# Autodesk Inventor assembly: body_new
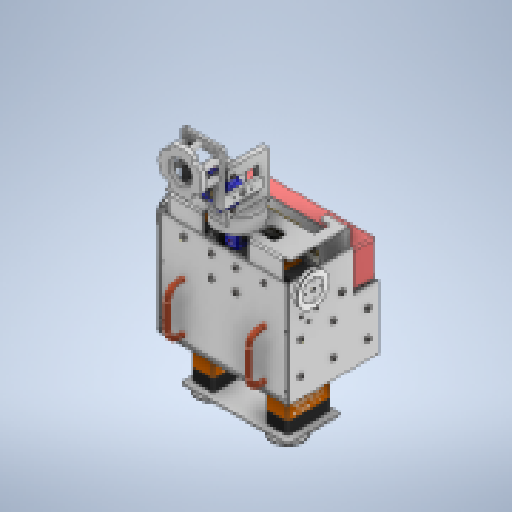
[picture p0: Inventor's stored thumbnail of the model, 512x512]
Saved by Autodesk Inventor 2027.1 (Build 311270010, 270A)
## iProperties
Created: 2025-05-30
Part Number: body_new
Document SubType Name: Assembly
Designer: chris
Author: chris
## Documents named in this file (30)
- C:\Users\chanh\Documents\RHp_Humanoid_ver1\Total\body_new.iam
- C:\Users\chanh\Documents\RHp_Humanoid_ver1\Part_Body\Frame\Body\body_main_frame.ipt
- C:\Users\chanh\Documents\RHp_Humanoid_ver1\Part_Body\Frame\Body\body_back_frame.ipt
- C:\Users\chanh\Documents\RHp_Humanoid_ver1\Part_Body\Frame\Body\body_front_frame.ipt
- C:\Users\chanh\Documents\RHp_Humanoid_ver1\Part_Body\Frame\Body\body_middle_frame.ipt
- C:\Users\chanh\Documents\RHp_Humanoid_ver1\Part_Body\Frame\Body\body_motor_L_frame.ipt
- C:\Users\chanh\Documents\RHp_Humanoid_ver1\Part_Body\Frame\Body\body_motor_R_frame.ipt
- C:\Users\chanh\Documents\RHp_Humanoid_ver1\Part_Body\Other Parts\Servo_Driver.ipt
- C:\Users\chanh\Documents\RHp_Humanoid_ver1\Part_Body\Other Parts\Battery_Pack.ipt
- C:\Users\chanh\Documents\RHp_Humanoid_ver1\Part_Body\Other Parts\jetson_orin_super.ipt
- C:\Users\chanh\Documents\RHp_Humanoid_ver1\Part_Body\Frame\Body\body_bottom_frame.ipt
- C:\Users\chanh\Documents\RHp_Humanoid_ver1\Part_Body\Other Parts\frame_motor_support_top_R.ipt
- C:\Users\chanh\Documents\RHp_Humanoid_ver1\Part_Body\Other Parts\frame_motor_support_top_L.ipt
- C:\Users\chanh\Documents\RHp_Humanoid_ver1\Part_Body\Bolt, Bearing, Nut, Washer\2030 Teflon Sheet.ipt
- C:\Users\chanh\Documents\RHp_Humanoid_ver1\Part_Body\Other Parts\frame_support.ipt
- C:\Users\chanh\Documents\RHp_Humanoid_ver1\Part_Body\HTD-45H, Horn (Silver)\HTD-45H\HTD-45H.ipt
- C:\Users\chanh\Documents\RHp_Humanoid_ver1\Part_Body\Other Parts\frame_motor_support_bottom_L.ipt
- C:\Users\chanh\Documents\RHp_Humanoid_ver1\Part_Body\Other Parts\frame_motor_support_bottom_R.ipt
- C:\Users\chanh\Documents\RHp_Humanoid_ver1\Part_Body\Bolt, Bearing, Nut, Washer\M3x6 Bolt.ipt
- C:\Users\chanh\Documents\RHp_Humanoid_ver1\Part_Body\Bolt, Bearing, Nut, Washer\M3 Nut.ipt
- C:\Users\chanh\Documents\RHp_Humanoid_ver1\Part_Body\Bolt, Bearing, Nut, Washer\M2x4 Bolt.ipt
- C:\Users\chanh\Documents\RHp_Humanoid_ver1\Part_Body\Bolt, Bearing, Nut, Washer\M2x6 Bolt.ipt
- C:\Users\chanh\Documents\RHp_Humanoid_ver1\Part_Body\Bolt, Bearing, Nut, Washer\M2x35 Bolt.ipt
- C:\Users\chanh\Documents\RHp_Humanoid_ver1\Part_Body\HTD-45H, Horn (Silver)\HTD-45H\M2x32.ipt
- C:\Users\chanh\Documents\RHp_Humanoid_ver1\Part_Body\HTD-45H, Horn (Silver)\Horn\Top Horn.ipt
- C:\Users\chanh\Documents\RHp_Humanoid_ver1\Part_Body\Frame\Body\body_top_frame2.ipt
- C:\Users\chanh\Documents\RHp_Humanoid_ver1\Part_Body\Other Parts\head\SG90 - Micro Servo 9g - Tower Pro\SG90 - Micro Servo 9g - Tower Pro\SG90 - Micro Servo 9g - Tower Pro - bottom.iam
- C:\Users\chanh\Documents\RHp_Humanoid_ver1\Part_Body\Other Parts\head\head_bottom.ipt
- C:\Users\chanh\Documents\RHp_Humanoid_ver1\Part_Body\Other Parts\head\head_top.ipt
- C:\Users\chanh\Documents\RHp_Humanoid_ver1\Part_Body\Other Parts\head\SG90 - Micro Servo 9g - Tower Pro\SG90 - Micro Servo 9g - Tower Pro\SG90 - Micro Servo 9g - Tower Pro - top.iam
## Components (171 placed, 29 different names)
1. head_bottom:1 — Rigid:157, Mate:93, Mate:94, Flush:38
2. head_top:1 — Rigid:158
3. SG90 - Micro Servo 9g - Tower Pro - top:1 [sub-assembly] — Mate:93, Mate:94, Flush:38, Rigid:158
4. body_main_frame:1 — Mate:3, Flush:2, Mate:4, Mate:5, Flush:3, Flush:4, Mate:6, Flush:5, Mate:8, Mate:10, Mate:16, Mate:18, Flush:13, Mate:30, Flush:30, Flush:31, Mate:46, Mate:47, Mate:48, Mate:49, Mate:50, Mate:51, Mate:64, Mate:66, Mate:68, Flush:34, Flush:35, Mate:69, Flush:36, Flush:37, Rigid:25, Rigid:26, Rigid:29, Rigid:30, Rigid:33, Rigid:34, Rigid:35, Rigid:36, Rigid:65, Rigid:66, Rigid:67, Rigid:68, Rigid:73, Rigid:74, Rigid:75, Rigid:76, Rigid:77, Rigid:78, Rigid:99, Rigid:100, Rigid:101, Rigid:102, Rigid:103, Rigid:104, Rigid:105, Rigid:106, Rigid:107, Rigid:108, Rigid:109, Rigid:110, Rigid:145, Rigid:147
5. body_middle_frame:1 — Mate:6, Flush:5, Flush:6, Mate:17, Mate:28, Flush:29, Mate:29, Mate:65, Flush:32, Flush:33, Mate:67, Rigid:9, Rigid:10, Rigid:11, Rigid:12, Rigid:13, Rigid:14, Rigid:15, Rigid:16, Rigid:27, Rigid:28, Rigid:31, Rigid:32
6. body_front_frame:1 — Mate:5, Flush:3, Flush:4, Flush:6, Mate:7, Flush:7, Mate:9, Flush:8, Mate:58, Mate:59, Mate:60, Mate:61, Mate:62, Mate:63, Rigid:17, Rigid:18, Rigid:19, Rigid:20, Rigid:49, Rigid:50, Rigid:51, Rigid:52, Rigid:57, Rigid:58, Rigid:59, Rigid:60, Rigid:69, Rigid:70, Rigid:71, Rigid:72, Rigid:149, Rigid:151, Rigid:152
7. body_back_frame:1 — Mate:3, Flush:2, Mate:4, Mate:19, Mate:52, Mate:53, Mate:54, Mate:55, Mate:56, Mate:57, Rigid:37, Rigid:38, Rigid:39, Rigid:40, Rigid:61, Rigid:62, Rigid:63, Rigid:64
8. body_top_frame2:1 — Rigid:152, Rigid:153, Rigid:154, Rigid:155, Rigid:156, Mate:89, Mate:91, Mate:95, Mate:96
9. body_bottom_frame:1 — Mate:80, Mate:81, Mate:82, Mate:83, Mate:84, Mate:85, Mate:86, Mate:87, Mate:88, Rigid:111, Rigid:112, Rigid:113, Rigid:114, Rigid:115, Rigid:116
10. Servo_Driver:1 — Mate:16, Mate:17, Mate:18, Rigid:1, Rigid:2, Rigid:3, Rigid:4
11. Battery_Pack:1 — Mate:19, Flush:13, Mate:89
12. jetson_orin_super:1 — Mate:28, Flush:29, Mate:29
13. SG90 - Micro Servo 9g - Tower Pro - bottom:1 [sub-assembly] — Mate:91, Rigid:157, Mate:95, Mate:96
14. HTD-45H:1 — Mate:69, Flush:36, Flush:37, Mate:81, Rigid:127, Rigid:128, Rotational:8
15. HTD-45H:2 — Mate:68, Flush:34, Flush:35, Mate:80, Mate:82, Rigid:125, Rigid:126, Rotational:7
16. HTD-45H:3 — Mate:66, Flush:33, Mate:67, Rigid:129, Rigid:130, Rotational:5
17. HTD-45H:4 — Mate:64, Mate:65, Flush:32, Rigid:131, Rigid:132, Rotational:6
18. Top Horn:5 — Rotational:5
19. Top Horn:7 — Rotational:6
20. 2030 Teflon Sheet:1 — Insert:2, Insert:9
21. 2030 Teflon Sheet:2 — Insert:2
22. 2030 Teflon Sheet:3 — Insert:4, Insert:10
23. 2030 Teflon Sheet:4 — Insert:4
24. frame_motor_support_top_R:1 — Mate:46, Mate:47, Mate:48, Rigid:81, Rigid:84, Rigid:85, Rigid:86, Insert:10
25. frame_motor_support_top_L:1 — Mate:49, Mate:50, Mate:51, Rigid:79, Rigid:80, Rigid:82, Rigid:83, Insert:9
26. body_motor_R_frame:1 — Mate:9, Mate:10, Flush:8, Rigid:5, Rigid:7, Rigid:22, Rigid:24, Rigid:53, Rigid:54, Rigid:87, Rigid:88, Rigid:89, Rigid:90, Rigid:91, Rigid:92
27. body_motor_L_frame:1 — Mate:7, Flush:7, Mate:8, Rigid:6, Rigid:8, Rigid:21, Rigid:23, Rigid:55, Rigid:56, Rigid:93, Rigid:94, Rigid:95, Rigid:96, Rigid:97, Rigid:98
28. M3x6 Bolt:9 — Rigid:17
29. M3x6 Bolt:10 — Rigid:20
30. M3x6 Bolt:11 — Rigid:18
31. M3x6 Bolt:12 — Rigid:19
32. M3x6 Bolt:13 — Rigid:29
33. M3x6 Bolt:14 — Rigid:30
34. M3x6 Bolt:15 — Rigid:26
35. M3x6 Bolt:16 — Rigid:25
36. M3 Nut:9 — Rigid:24
37. M3 Nut:10 — Rigid:23
38. M3 Nut:11 — Rigid:22
39. M3 Nut:12 — Rigid:21
40. M3 Nut:13 — Rigid:31
41. M3 Nut:14 — Rigid:32
42. M3 Nut:15 — Rigid:27
43. M3 Nut:16 — Rigid:28
44. M3x6 Bolt:1 — Rigid:4
45. M3x6 Bolt:2 — Rigid:3
46. M3x6 Bolt:3 — Rigid:2
47. M3x6 Bolt:4 — Rigid:1
48. M3x6 Bolt:5 — Rigid:5
49. M3x6 Bolt:6 — Rigid:6
50. M3x6 Bolt:7 — Rigid:7
51. M3x6 Bolt:8 — Rigid:8
52. M3 Nut:1 — Rigid:9
53. M3 Nut:2 — Rigid:10
54. M3 Nut:3 — Rigid:11
55. M3 Nut:4 — Rigid:12
56. M3 Nut:5 — Rigid:13
57. M3 Nut:6 — Rigid:14
58. M3 Nut:7 — Rigid:15
59. M3 Nut:8 — Rigid:16
60. frame_support:3 — Mate:59, Mate:61, Mate:63
61. frame_support:4 — Mate:58, Mate:60, Mate:62
62. M3x6 Bolt:37 — Rigid:66
63. M3x6 Bolt:38 — Rigid:65
64. M3x6 Bolt:39 — Rigid:68
65. M3x6 Bolt:40 — Rigid:67
66. M3 Nut:29 — Rigid:69
67. M3 Nut:30 — Rigid:70
68. M3 Nut:31 — Rigid:71
69. M3 Nut:32 — Rigid:72
70. M3x6 Bolt:29 — Rigid:57
71. M3x6 Bolt:30 — Rigid:58
72. M3x6 Bolt:31 — Rigid:60
73. M3x6 Bolt:32 — Rigid:59
74. M3x6 Bolt:25 — Rigid:49
75. M3x6 Bolt:26 — Rigid:51
76. M3x6 Bolt:27 — Rigid:50
77. M3x6 Bolt:28 — Rigid:52
78. M3 Nut:25 — Rigid:53
79. M3 Nut:26 — Rigid:55
80. M3 Nut:27 — Rigid:54
81. M3 Nut:28 — Rigid:56
82. frame_support:1 — Mate:52, Mate:53, Mate:54
83. frame_support:2 — Mate:55, Mate:56, Mate:57
84. M3x6 Bolt:33 — Rigid:61
85. M3x6 Bolt:34 — Rigid:62
86. M3x6 Bolt:35 — Rigid:64
87. M3x6 Bolt:36 — Rigid:63
88. M3x6 Bolt:17 — Rigid:33
89. M3x6 Bolt:18 — Rigid:35
90. M3x6 Bolt:19 — Rigid:34
91. M3x6 Bolt:20 — Rigid:36
92. M3 Nut:17 — Rigid:37
93. M3 Nut:18 — Rigid:38
94. M3 Nut:19 — Rigid:39
95. M3 Nut:20 — Rigid:40
96. M3x6 Bolt:45 — Rigid:147
97. M3x6 Bolt:46 — Rigid:151
98. M3x6 Bolt:47 — Rigid:145
99. M3x6 Bolt:48 — Rigid:149
100. M3 Nut:41 — Rigid:156
101. M3 Nut:42 — Rigid:153
102. M3 Nut:43 — Rigid:155
103. M3 Nut:44 — Rigid:154
104. frame_motor_support_bottom_R:1 — Mate:83, Mate:84, Mate:85, Rigid:119, Rigid:120, Rigid:121, Rigid:122, Insert:12
105. frame_motor_support_bottom_L:1 — Mate:86, Mate:87, Mate:88, Rigid:117, Rigid:118, Rigid:123, Rigid:124, Insert:11
106. 2030 Teflon Sheet:5 — Insert:8
107. 2030 Teflon Sheet:6 — Insert:8, Insert:11
108. 2030 Teflon Sheet:7 — Insert:6
109. 2030 Teflon Sheet:8 — Insert:6, Insert:12
110. Top Horn:6 — Rotational:7
111. Top Horn:8 — Rotational:8
112. M2x32:7 — Rigid:132
113. M2x32:8 — Rigid:131
114. M2x4 Bolt:7 — Rigid:87
115. M2x4 Bolt:8 — Rigid:89
116. M2x4 Bolt:9 — Rigid:91
117. M2x4 Bolt:10 — Rigid:88
118. M2x4 Bolt:11 — Rigid:90
119. M2x4 Bolt:12 — Rigid:92
120. M2x4 Bolt:4 — Rigid:77
121. M2x4 Bolt:5 — Rigid:78
122. M2x4 Bolt:6 — Rigid:76
123. M2x6 Bolt:3 — Rigid:81
124. M2x6 Bolt:4 — Rigid:86
125. M2x35 Bolt:3 — Rigid:84
126. M2x35 Bolt:4 — Rigid:85
127. M2x32:5 — Rigid:130
128. M2x32:6 — Rigid:129
129. M2x4 Bolt:13 — Rigid:93
130. M2x4 Bolt:14 — Rigid:98
131. M2x4 Bolt:15 — Rigid:97
132. M2x4 Bolt:16 — Rigid:94
133. M2x4 Bolt:17 — Rigid:95
134. M2x4 Bolt:18 — Rigid:96
135. M2x4 Bolt:1 — Rigid:73
136. M2x4 Bolt:2 — Rigid:74
137. M2x4 Bolt:3 — Rigid:75
138. M2x6 Bolt:1 — Rigid:79
139. M2x6 Bolt:2 — Rigid:80
140. M2x35 Bolt:1 — Rigid:82
141. M2x35 Bolt:2 — Rigid:83
142. M2x32:1 — Rigid:126
143. M2x32:2 — Rigid:125
144. M2x4 Bolt:34 — Rigid:114
145. M2x4 Bolt:35 — Rigid:116
146. M2x4 Bolt:36 — Rigid:115
147. M2x6 Bolt:7 — Rigid:119
148. M2x6 Bolt:8 — Rigid:120
149. M2x35 Bolt:5 — Rigid:121
150. M2x35 Bolt:6 — Rigid:122
151. M2x4 Bolt:19 — Rigid:99
152. M2x4 Bolt:20 — Rigid:100
153. M2x4 Bolt:21 — Rigid:101
154. M2x4 Bolt:22 — Rigid:104
155. M2x4 Bolt:23 — Rigid:103
156. M2x4 Bolt:24 — Rigid:102
157. M2x32:3 — Rigid:127
158. M2x32:4 — Rigid:128
159. M2x4 Bolt:31 — Rigid:111
160. M2x4 Bolt:32 — Rigid:112
161. M2x4 Bolt:33 — Rigid:113
162. M2x6 Bolt:5 — Rigid:117
163. M2x6 Bolt:6 — Rigid:118
164. M2x35 Bolt:7 — Rigid:123
165. M2x35 Bolt:8 — Rigid:124
166. M2x4 Bolt:25 — Rigid:110
167. M2x4 Bolt:26 — Rigid:109
168. M2x4 Bolt:27 — Rigid:108
169. M2x4 Bolt:28 — Rigid:107
170. M2x4 Bolt:29 — Rigid:106
171. M2x4 Bolt:30 — Rigid:105
## Relationships (219: WeldJoint 135, Mate 54, Flush 18, Insert 8, RevoluteJoint 4)
- Mate:3: body_main_frame:1 ↔ body_back_frame:1
- Flush:2: body_main_frame:1 ↔ body_back_frame:1
- Mate:4 (2 mm): body_main_frame:1 ↔ body_back_frame:1
- Mate:5: body_main_frame:1 ↔ body_front_frame:1
- Flush:3 (1.5 mm): body_main_frame:1 ↔ body_front_frame:1
- Flush:4: body_main_frame:1 ↔ body_front_frame:1
- Mate:6: body_main_frame:1 ↔ body_middle_frame:1
- Flush:5 (1.5 mm): body_main_frame:1 ↔ body_middle_frame:1
- Flush:6 (-30 mm): body_middle_frame:1 ↔ body_front_frame:1
- Mate:7: body_front_frame:1 ↔ body_motor_L_frame:1
- Flush:7: body_front_frame:1 ↔ body_motor_L_frame:1
- Mate:8 (40 mm): body_main_frame:1 ↔ body_motor_L_frame:1
- Mate:9: body_front_frame:1 ↔ body_motor_R_frame:1
- Mate:10 (40 mm): body_main_frame:1 ↔ body_motor_R_frame:1
- Flush:8: body_front_frame:1 ↔ body_motor_R_frame:1
- Mate:16 (10 mm): body_main_frame:1 ↔ Servo_Driver:1
- Mate:17: body_middle_frame:1 ↔ Servo_Driver:1
- Mate:18 (31 mm): body_main_frame:1 ↔ Servo_Driver:1
- Mate:19: body_back_frame:1 ↔ Battery_Pack:1
- Flush:13 (-2.5 mm): body_main_frame:1 ↔ Battery_Pack:1
- Mate:28: body_middle_frame:1 ↔ jetson_orin_super:1
- Flush:29 (4 mm): body_middle_frame:1 ↔ jetson_orin_super:1
- Mate:29 (7 mm): body_middle_frame:1 ↔ jetson_orin_super:1
- Mate:30: body_main_frame:1
- Flush:30: body_main_frame:1
- Flush:31: body_main_frame:1
- Mate:46: body_main_frame:1 ↔ frame_motor_support_top_R:1
- Mate:47: body_main_frame:1 ↔ frame_motor_support_top_R:1
- Mate:48: body_main_frame:1 ↔ frame_motor_support_top_R:1
- Mate:49: body_main_frame:1 ↔ frame_motor_support_top_L:1
- Mate:50: body_main_frame:1 ↔ frame_motor_support_top_L:1
- Mate:51: body_main_frame:1 ↔ frame_motor_support_top_L:1
- Insert:2 (0.07 mm): 2030 Teflon Sheet:1 ↔ 2030 Teflon Sheet:2
- Insert:4 (0.07 mm): 2030 Teflon Sheet:3 ↔ 2030 Teflon Sheet:4
- Mate:52: body_back_frame:1 ↔ frame_support:1
- Mate:53: body_back_frame:1 ↔ frame_support:1
- Mate:54: body_back_frame:1 ↔ frame_support:1
- Mate:55: body_back_frame:1 ↔ frame_support:2
- Mate:56: body_back_frame:1 ↔ frame_support:2
- Mate:57: body_back_frame:1 ↔ frame_support:2
- Mate:58: body_front_frame:1 ↔ frame_support:4
- Mate:59: body_front_frame:1 ↔ frame_support:3
- Mate:60: body_front_frame:1 ↔ frame_support:4
- Mate:61: body_front_frame:1 ↔ frame_support:3
- Mate:62: body_front_frame:1 ↔ frame_support:4
- Mate:63: body_front_frame:1 ↔ frame_support:3
- Mate:64: body_main_frame:1 ↔ HTD-45H:4
- Mate:65 (2 mm): body_middle_frame:1 ↔ HTD-45H:4
- Flush:32: body_middle_frame:1 ↔ HTD-45H:4
- Mate:66: body_main_frame:1 ↔ HTD-45H:3
- Flush:33: body_middle_frame:1 ↔ HTD-45H:3
- Mate:67 (2 mm): body_middle_frame:1 ↔ HTD-45H:3
- Mate:68: body_main_frame:1 ↔ HTD-45H:2
- Flush:34 (15 mm): body_main_frame:1 ↔ HTD-45H:2
- Flush:35 (16.5 mm): body_main_frame:1 ↔ HTD-45H:2
- Mate:69: body_main_frame:1 ↔ HTD-45H:1
- Flush:36 (15 mm): body_main_frame:1 ↔ HTD-45H:1
- Flush:37 (16.5 mm): body_main_frame:1 ↔ HTD-45H:1
- Mate:80: body_bottom_frame:1 ↔ HTD-45H:2
- Mate:81: body_bottom_frame:1 ↔ HTD-45H:1
- Mate:82: body_bottom_frame:1 ↔ HTD-45H:2
- Mate:83: body_bottom_frame:1 ↔ frame_motor_support_bottom_R:1
- Mate:84: body_bottom_frame:1 ↔ frame_motor_support_bottom_R:1
- Mate:85: body_bottom_frame:1 ↔ frame_motor_support_bottom_R:1
- Mate:86: body_bottom_frame:1 ↔ frame_motor_support_bottom_L:1
- Mate:87: body_bottom_frame:1 ↔ frame_motor_support_bottom_L:1
- Mate:88: body_bottom_frame:1 ↔ frame_motor_support_bottom_L:1
- Insert:6 (0.07 mm): 2030 Teflon Sheet:7 ↔ 2030 Teflon Sheet:8
- Insert:8 (0.07 mm): 2030 Teflon Sheet:5 ↔ 2030 Teflon Sheet:6
- Rigid:1 [WeldJoint]: Servo_Driver:1 ↔ M3x6 Bolt:4
- Rigid:2 [WeldJoint]: Servo_Driver:1 ↔ M3x6 Bolt:3
- Rigid:3 [WeldJoint]: Servo_Driver:1 ↔ M3x6 Bolt:2
- Rigid:4 [WeldJoint]: Servo_Driver:1 ↔ M3x6 Bolt:1
- Rigid:5 [WeldJoint]: body_motor_R_frame:1 ↔ M3x6 Bolt:5
- Rigid:6 [WeldJoint]: body_motor_L_frame:1 ↔ M3x6 Bolt:6
- Rigid:7 [WeldJoint]: body_motor_R_frame:1 ↔ M3x6 Bolt:7
- Rigid:8 [WeldJoint]: body_motor_L_frame:1 ↔ M3x6 Bolt:8
- Rigid:9 [WeldJoint]: body_middle_frame:1 ↔ M3 Nut:1
- Rigid:10 [WeldJoint]: body_middle_frame:1 ↔ M3 Nut:2
- Rigid:11 [WeldJoint]: body_middle_frame:1 ↔ M3 Nut:3
- Rigid:12 [WeldJoint]: body_middle_frame:1 ↔ M3 Nut:4
- Rigid:13 [WeldJoint]: body_middle_frame:1 ↔ M3 Nut:5
- Rigid:14 [WeldJoint]: body_middle_frame:1 ↔ M3 Nut:6
- Rigid:15 [WeldJoint]: body_middle_frame:1 ↔ M3 Nut:7
- Rigid:16 [WeldJoint]: body_middle_frame:1 ↔ M3 Nut:8
- Rigid:17 [WeldJoint]: body_front_frame:1 ↔ M3x6 Bolt:9
- Rigid:18 [WeldJoint]: body_front_frame:1 ↔ M3x6 Bolt:11
- Rigid:19 [WeldJoint]: body_front_frame:1 ↔ M3x6 Bolt:12
- Rigid:20 [WeldJoint]: body_front_frame:1 ↔ M3x6 Bolt:10
- Rigid:21 [WeldJoint]: body_motor_L_frame:1 ↔ M3 Nut:12
- Rigid:22 [WeldJoint]: body_motor_R_frame:1 ↔ M3 Nut:11
- Rigid:23 [WeldJoint]: body_motor_L_frame:1 ↔ M3 Nut:10
- Rigid:24 [WeldJoint]: body_motor_R_frame:1 ↔ M3 Nut:9
- Rigid:25 [WeldJoint]: body_main_frame:1 ↔ M3x6 Bolt:16
- Rigid:26 [WeldJoint]: body_main_frame:1 ↔ M3x6 Bolt:15
- Rigid:27 [WeldJoint]: body_middle_frame:1 ↔ M3 Nut:15
- Rigid:28 [WeldJoint]: body_middle_frame:1 ↔ M3 Nut:16
- Rigid:29 [WeldJoint]: body_main_frame:1 ↔ M3x6 Bolt:13
- Rigid:30 [WeldJoint]: body_main_frame:1 ↔ M3x6 Bolt:14
- Rigid:31 [WeldJoint]: body_middle_frame:1 ↔ M3 Nut:13
- Rigid:32 [WeldJoint]: body_middle_frame:1 ↔ M3 Nut:14
- Rigid:33 [WeldJoint]: body_main_frame:1 ↔ M3x6 Bolt:17
- Rigid:34 [WeldJoint]: body_main_frame:1 ↔ M3x6 Bolt:19
- Rigid:35 [WeldJoint]: body_main_frame:1 ↔ M3x6 Bolt:18
- Rigid:36 [WeldJoint]: body_main_frame:1 ↔ M3x6 Bolt:20
- Rigid:37 [WeldJoint]: body_back_frame:1 ↔ M3 Nut:17
- Rigid:38 [WeldJoint]: body_back_frame:1 ↔ M3 Nut:18
- Rigid:39 [WeldJoint]: body_back_frame:1 ↔ M3 Nut:19
- Rigid:40 [WeldJoint]: body_back_frame:1 ↔ M3 Nut:20
- Rigid:49 [WeldJoint]: body_front_frame:1 ↔ M3x6 Bolt:25
- Rigid:50 [WeldJoint]: body_front_frame:1 ↔ M3x6 Bolt:27
- Rigid:51 [WeldJoint]: body_front_frame:1 ↔ M3x6 Bolt:26
- Rigid:52 [WeldJoint]: body_front_frame:1 ↔ M3x6 Bolt:28
- Rigid:53 [WeldJoint]: body_motor_R_frame:1 ↔ M3 Nut:25
- Rigid:54 [WeldJoint]: body_motor_R_frame:1 ↔ M3 Nut:27
- Rigid:55 [WeldJoint]: body_motor_L_frame:1 ↔ M3 Nut:26
- Rigid:56 [WeldJoint]: body_motor_L_frame:1 ↔ M3 Nut:28
- Rigid:57 [WeldJoint]: body_front_frame:1 ↔ M3x6 Bolt:29
- Rigid:58 [WeldJoint]: body_front_frame:1 ↔ M3x6 Bolt:30
- Rigid:59 [WeldJoint]: body_front_frame:1 ↔ M3x6 Bolt:32
- Rigid:60 [WeldJoint]: body_front_frame:1 ↔ M3x6 Bolt:31
- Rigid:61 [WeldJoint]: body_back_frame:1 ↔ M3x6 Bolt:33
- Rigid:62 [WeldJoint]: body_back_frame:1 ↔ M3x6 Bolt:34
- Rigid:63 [WeldJoint]: body_back_frame:1 ↔ M3x6 Bolt:36
- Rigid:64 [WeldJoint]: body_back_frame:1 ↔ M3x6 Bolt:35
- Rigid:65 [WeldJoint]: body_main_frame:1 ↔ M3x6 Bolt:38
- Rigid:66 [WeldJoint]: body_main_frame:1 ↔ M3x6 Bolt:37
- Rigid:67 [WeldJoint]: body_main_frame:1 ↔ M3x6 Bolt:40
- Rigid:68 [WeldJoint]: body_main_frame:1 ↔ M3x6 Bolt:39
- Rigid:69 [WeldJoint]: body_front_frame:1 ↔ M3 Nut:29
- Rigid:70 [WeldJoint]: body_front_frame:1 ↔ M3 Nut:30
- Rigid:71 [WeldJoint]: body_front_frame:1 ↔ M3 Nut:31
- Rigid:72 [WeldJoint]: body_front_frame:1 ↔ M3 Nut:32
- Rigid:73 [WeldJoint]: body_main_frame:1 ↔ M2x4 Bolt:1
- Rigid:74 [WeldJoint]: body_main_frame:1 ↔ M2x4 Bolt:2
- Rigid:75 [WeldJoint]: body_main_frame:1 ↔ M2x4 Bolt:3
- Rigid:76 [WeldJoint]: body_main_frame:1 ↔ M2x4 Bolt:6
- Rigid:77 [WeldJoint]: body_main_frame:1 ↔ M2x4 Bolt:4
- Rigid:78 [WeldJoint]: body_main_frame:1 ↔ M2x4 Bolt:5
- Rigid:79 [WeldJoint]: frame_motor_support_top_L:1 ↔ M2x6 Bolt:1
- Rigid:80 [WeldJoint]: frame_motor_support_top_L:1 ↔ M2x6 Bolt:2
- Rigid:81 [WeldJoint]: frame_motor_support_top_R:1 ↔ M2x6 Bolt:3
- Rigid:82 [WeldJoint]: frame_motor_support_top_L:1 ↔ M2x35 Bolt:1
- Rigid:83 [WeldJoint]: frame_motor_support_top_L:1 ↔ M2x35 Bolt:2
- Rigid:84 [WeldJoint]: frame_motor_support_top_R:1 ↔ M2x35 Bolt:3
- Rigid:85 [WeldJoint]: frame_motor_support_top_R:1 ↔ M2x35 Bolt:4
- Rigid:86 [WeldJoint]: frame_motor_support_top_R:1 ↔ M2x6 Bolt:4
- Rigid:87 [WeldJoint]: body_motor_R_frame:1 ↔ M2x4 Bolt:7
- Rigid:88 [WeldJoint]: body_motor_R_frame:1 ↔ M2x4 Bolt:10
- Rigid:89 [WeldJoint]: body_motor_R_frame:1 ↔ M2x4 Bolt:8
- Rigid:90 [WeldJoint]: body_motor_R_frame:1 ↔ M2x4 Bolt:11
- Rigid:91 [WeldJoint]: body_motor_R_frame:1 ↔ M2x4 Bolt:9
- Rigid:92 [WeldJoint]: body_motor_R_frame:1 ↔ M2x4 Bolt:12
- Rigid:93 [WeldJoint]: body_motor_L_frame:1 ↔ M2x4 Bolt:13
- Rigid:94 [WeldJoint]: body_motor_L_frame:1 ↔ M2x4 Bolt:16
- Rigid:95 [WeldJoint]: body_motor_L_frame:1 ↔ M2x4 Bolt:17
- Rigid:96 [WeldJoint]: body_motor_L_frame:1 ↔ M2x4 Bolt:18
- Rigid:97 [WeldJoint]: body_motor_L_frame:1 ↔ M2x4 Bolt:15
- Rigid:98 [WeldJoint]: body_motor_L_frame:1 ↔ M2x4 Bolt:14
- Rigid:99 [WeldJoint]: body_main_frame:1 ↔ M2x4 Bolt:19
- Rigid:100 [WeldJoint]: body_main_frame:1 ↔ M2x4 Bolt:20
- Rigid:101 [WeldJoint]: body_main_frame:1 ↔ M2x4 Bolt:21
- Rigid:102 [WeldJoint]: body_main_frame:1 ↔ M2x4 Bolt:24
- Rigid:103 [WeldJoint]: body_main_frame:1 ↔ M2x4 Bolt:23
- Rigid:104 [WeldJoint]: body_main_frame:1 ↔ M2x4 Bolt:22
- Rigid:105 [WeldJoint]: body_main_frame:1 ↔ M2x4 Bolt:30
- Rigid:106 [WeldJoint]: body_main_frame:1 ↔ M2x4 Bolt:29
- Rigid:107 [WeldJoint]: body_main_frame:1 ↔ M2x4 Bolt:28
- Rigid:108 [WeldJoint]: body_main_frame:1 ↔ M2x4 Bolt:27
- Rigid:109 [WeldJoint]: body_main_frame:1 ↔ M2x4 Bolt:26
- Rigid:110 [WeldJoint]: body_main_frame:1 ↔ M2x4 Bolt:25
- Rigid:111 [WeldJoint]: body_bottom_frame:1 ↔ M2x4 Bolt:31
- Rigid:112 [WeldJoint]: body_bottom_frame:1 ↔ M2x4 Bolt:32
- Rigid:113 [WeldJoint]: body_bottom_frame:1 ↔ M2x4 Bolt:33
- Rigid:114 [WeldJoint]: body_bottom_frame:1 ↔ M2x4 Bolt:34
- Rigid:115 [WeldJoint]: body_bottom_frame:1 ↔ M2x4 Bolt:36
- Rigid:116 [WeldJoint]: body_bottom_frame:1 ↔ M2x4 Bolt:35
- Rigid:117 [WeldJoint]: frame_motor_support_bottom_L:1 ↔ M2x6 Bolt:5
- Rigid:118 [WeldJoint]: frame_motor_support_bottom_L:1 ↔ M2x6 Bolt:6
- Rigid:119 [WeldJoint]: frame_motor_support_bottom_R:1 ↔ M2x6 Bolt:7
- Rigid:120 [WeldJoint]: frame_motor_support_bottom_R:1 ↔ M2x6 Bolt:8
- Rigid:121 [WeldJoint]: frame_motor_support_bottom_R:1 ↔ M2x35 Bolt:5
- Rigid:122 [WeldJoint]: frame_motor_support_bottom_R:1 ↔ M2x35 Bolt:6
- Rigid:123 [WeldJoint]: frame_motor_support_bottom_L:1 ↔ M2x35 Bolt:7
- Rigid:124 [WeldJoint]: frame_motor_support_bottom_L:1 ↔ M2x35 Bolt:8
- Rigid:125 [WeldJoint]: HTD-45H:2 ↔ M2x32:2
- Rigid:126 [WeldJoint]: HTD-45H:2 ↔ M2x32:1
- Rigid:127 [WeldJoint]: HTD-45H:1 ↔ M2x32:3
- Rigid:128 [WeldJoint]: HTD-45H:1 ↔ M2x32:4
- Rigid:129 [WeldJoint]: HTD-45H:3 ↔ M2x32:6
- Rigid:130 [WeldJoint]: HTD-45H:3 ↔ M2x32:5
- Rigid:131 [WeldJoint]: HTD-45H:4 ↔ M2x32:8
- Rigid:132 [WeldJoint]: HTD-45H:4 ↔ M2x32:7
- Rigid:145 [WeldJoint]: body_main_frame:1 ↔ M3x6 Bolt:47
- Rigid:147 [WeldJoint]: body_main_frame:1 ↔ M3x6 Bolt:45
- Rigid:149 [WeldJoint]: body_front_frame:1 ↔ M3x6 Bolt:48
- Rigid:151 [WeldJoint]: body_front_frame:1 ↔ M3x6 Bolt:46
- Rotational:5 [RevoluteJoint]: HTD-45H:3 ↔ Top Horn:5
- Rotational:6 [RevoluteJoint]: HTD-45H:4 ↔ Top Horn:7
- Rotational:7 [RevoluteJoint]: HTD-45H:2 ↔ Top Horn:6
- Rotational:8 [RevoluteJoint]: HTD-45H:1 ↔ Top Horn:8
- Insert:9: 2030 Teflon Sheet:1 ↔ frame_motor_support_top_L:1
- Insert:10: 2030 Teflon Sheet:3 ↔ frame_motor_support_top_R:1
- Insert:11: frame_motor_support_bottom_L:1 ↔ 2030 Teflon Sheet:6
- Insert:12: frame_motor_support_bottom_R:1 ↔ 2030 Teflon Sheet:8
- Rigid:152 [WeldJoint]: body_front_frame:1 ↔ body_top_frame2:1
- Rigid:153 [WeldJoint]: body_top_frame2:1 ↔ M3 Nut:42
- Rigid:154 [WeldJoint]: body_top_frame2:1 ↔ M3 Nut:44
- Rigid:155 [WeldJoint]: body_top_frame2:1 ↔ M3 Nut:43
- Rigid:156 [WeldJoint]: body_top_frame2:1 ↔ M3 Nut:41
- Mate:89: body_top_frame2:1 ↔ Battery_Pack:1
- Mate:91: body_top_frame2:1 ↔ SG90 - Micro Servo 9g - Tower Pro - bottom:1
- Rigid:157 [WeldJoint]: head_bottom:1 ↔ SG90 - Micro Servo 9g - Tower Pro - bottom:1
- Mate:93: head_bottom:1 ↔ SG90 - Micro Servo 9g - Tower Pro - top:1
- Mate:94 (0.25 mm): head_bottom:1 ↔ SG90 - Micro Servo 9g - Tower Pro - top:1
- Flush:38: head_bottom:1 ↔ SG90 - Micro Servo 9g - Tower Pro - top:1
- Rigid:158 [WeldJoint]: head_top:1 ↔ SG90 - Micro Servo 9g - Tower Pro - top:1
- Mate:95: body_top_frame2:1 ↔ SG90 - Micro Servo 9g - Tower Pro - bottom:1
- Mate:96: body_top_frame2:1 ↔ SG90 - Micro Servo 9g - Tower Pro - bottom:1
